# Autodesk Inventor assembly: Magnet Mount HSI
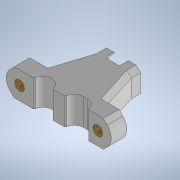
[picture p0: Inventor's stored thumbnail of the model, 180x180]
Saved by Autodesk Inventor 2022 (Build 260153000, 153)
## iProperties
Created: 2022-06-07
Part Number: Magnet Mount HSI
Document SubType Name: Assembly
Designer: Nick
Author: Nick
## Documents named in this file (3)
- Y:\Projects\Mini_Sand_Table\3D Printed\Models with Heat Set Inserts\Magnet Mount HSI.iam
- Y:\Projects\Mini_Sand_Table\3D Printed\Magnet Mount.ipt
- Y:\Projects\Bibble0\Hardware\M3 Heat Set Inserts.ipt
## Components (3 placed, 2 different names)
1. Magnet Mount:1 — Insert:1, Insert:2
2. M3 Heat Set Inserts:1 — Insert:1
3. M3 Heat Set Inserts:2 — Insert:2
## Relationships (2: Insert 2)
- Insert:1: Magnet Mount:1 ↔ M3 Heat Set Inserts:1
- Insert:2: Magnet Mount:1 ↔ M3 Heat Set Inserts:2
